# Autodesk Inventor assembly: YAxisMotor
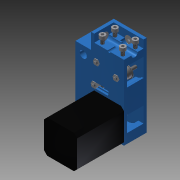
[picture p0: Inventor's stored thumbnail of the model, 180x180]
Saved by Autodesk Inventor 2015 (Build 190159000, 159)
## iProperties
Created: 2014-08-15
Part Number: YAxisMotor
Document SubType Name: Assembly
Designer: t_clevj
Author: t_clevj
## Documents named in this file (13)
- C:\Users\Jack\ownCloud\Projects\CoreXY\InventorModel\YAxis\YAxisMotor.iam
- C:\Users\Jack\ownCloud\Projects\CoreXY\InventorModel\YAxis\YAxisMotor\YMotorBlockLeft.ipt
- C:\Users\Jack\ownCloud\Projects\CoreXY\InventorModel\YAxis\YAxisMotor\YMotorCapLeft.ipt
- C:\Users\Jack\ownCloud\Projects\CoreXY\InventorModel\Hardware\Bolts\SHCS\SHCS4\SHCS4x30.ipt
- C:\Users\Jack\ownCloud\Projects\CoreXY\InventorModel\Hardware\Bolts\SHCS\SHCS3\SHCS3x8.ipt
- C:\Users\Jack\ownCloud\Projects\CoreXY\InventorModel\Hardware\Bolts\SHCS\SHCS5\SHCS5x10.ipt
- C:\Users\Jack\ownCloud\Projects\CoreXY\InventorModel\Hardware\Bearing\BearingRadialBall\BearingRadialBallF624zz.ipt
- C:\Users\Jack\ownCloud\Projects\CoreXY\InventorModel\Hardware\Wahsers\M4Washer.ipt
- C:\Users\Jack\ownCloud\Projects\CoreXY\InventorModel\Hardware\Nuts\Nut4.ipt
- C:\Users\Jack\ownCloud\Projects\CoreXY\InventorModel\Electronics\Motors\StepperMotorNema17.ipt
- C:\Users\Jack\ownCloud\Projects\CoreXY\InventorModel\Hardware\Bolts\SHCS\SHCS4\SHCS4x15.ipt
- C:\Users\Jack\ownCloud\Projects\CoreXY\InventorModel\Hardware\Bolts\FHS\FHS5\5x10FHS.ipt
- C:\Users\Jack\ownCloud\Projects\CoreXY\InventorModel\Hardware\Belt\PulleyGT2x20tx5mmBore.ipt
## Components (38 placed, 12 different names)
1. YMotorBlockLeft:1 — Mate:1, Mate:4, Flush:3, Mate:5, Mate:6, Mate:7, Mate:8, Slider:2, Mate:9, Mate:10, Mate:11, Mate:12, Mate:13, Mate:14, Mate:15, Mate:16, Mate:17, Mate:18, Mate:19, Mate:20, Mate:21, Mate:22, Mate:30, Mate:38, Mate:46, Angle:1, Mate:48, Angle:2, Mate:50, Angle:3, Mate:52, Mate:53, Mate:54, Angle:4, Angle:5, Angle:6, Angle:7, Mate:68, Mate:69, Mate:70, Mate:71, Mate:72, Mate:73, Flush:4, Flush:5, Mate:75
2. YMotorCapLeft:1 — Mate:1, Mate:6, Mate:56, Mate:57, Mate:58, Mate:59, Mate:60, Mate:61, Mate:62, Mate:63
3. SHCS4x30:3 — Mate:7, Mate:10, Mate:37, Mate:49
4. StepperMotorNema17:1 — Mate:53, Mate:54, Mate:55, Mate:74
5. 5x10FHS:1 — Mate:72, Flush:5
6. 5x10FHS:2 — Mate:73, Flush:4
7. PulleyGT2x20tx5mmBore:1 — Mate:74, Mate:75
8. Nut4:1 — Mate:47, Angle:1, Mate:48
9. Nut4:2 — Mate:49, Angle:2, Mate:50
10. Nut4:3 — Mate:51, Angle:3, Mate:52
11. M4Washer:1 — Mate:25, Mate:26
12. M4Washer:2 — Mate:27, Mate:28, Mate:29, Mate:30
13. M4Washer:3 — Mate:37
14. M4Washer:4 — Mate:38
15. M4Washer:5 — Mate:45
16. M4Washer:6 — Mate:46
17. SHCS4x30:5 — Slider:2, Mate:45, Mate:51
18. SHCS4x30:4 — Mate:8, Mate:9, Mate:29, Mate:47
19. BearingRadialBallF624zz:1 — Mate:23, Mate:24, Mate:25, Mate:26
20. BearingRadialBallF624zz:6 — Mate:23, Mate:24, Mate:27, Mate:28
21. BearingRadialBallF624zz:7
22. BearingRadialBallF624zz:8
23. BearingRadialBallF624zz:9
24. BearingRadialBallF624zz:10
25. SHCS5x10:2 — Mate:20, Mate:21
26. SHCS5x10:1 — Mate:19, Mate:22
27. SHCS3x8:3 — Mate:14, Mate:17
28. SHCS3x8:1 — Mate:12, Mate:18
29. SHCS3x8:2 — Mate:13, Mate:16
30. SHCS3x8:4 — Mate:11, Mate:15, Mate:55
31. SHCS4x15:1 — Mate:59, Mate:61, Mate:65
32. SHCS4x15:2 — Mate:58, Mate:62, Mate:67
33. SHCS4x15:3 — Mate:57, Mate:60, Mate:64
34. SHCS4x15:4 — Mate:56, Mate:63, Mate:66
35. Nut4:4 — Mate:66, Angle:6, Mate:70
36. Nut4:5 — Mate:67, Angle:7, Mate:71
37. Nut4:6 — Mate:64, Angle:5, Mate:69
38. Nut4:7 — Mate:65, Angle:4, Mate:68
## Relationships (84: Mate 73, Angle 7, Flush 3, TranslationJoint 1)
- Mate:1: YMotorBlockLeft:1 ↔ YMotorCapLeft:1
- Mate:4: YMotorBlockLeft:1
- Flush:3: YMotorBlockLeft:1
- Mate:5: YMotorBlockLeft:1
- Mate:6: YMotorBlockLeft:1 ↔ YMotorCapLeft:1
- Mate:7: YMotorBlockLeft:1 ↔ SHCS4x30:3
- Mate:8: YMotorBlockLeft:1 ↔ SHCS4x30:4
- Slider:2 [TranslationJoint]: YMotorBlockLeft:1 ↔ SHCS4x30:5
- Mate:9: YMotorBlockLeft:1 ↔ SHCS4x30:4
- Mate:10: YMotorBlockLeft:1 ↔ SHCS4x30:3
- Mate:11: YMotorBlockLeft:1 ↔ SHCS3x8:4
- Mate:12: YMotorBlockLeft:1 ↔ SHCS3x8:1
- Mate:13: YMotorBlockLeft:1 ↔ SHCS3x8:2
- Mate:14: YMotorBlockLeft:1 ↔ SHCS3x8:3
- Mate:15: YMotorBlockLeft:1 ↔ SHCS3x8:4
- Mate:16: YMotorBlockLeft:1 ↔ SHCS3x8:2
- Mate:17: YMotorBlockLeft:1 ↔ SHCS3x8:3
- Mate:18: YMotorBlockLeft:1 ↔ SHCS3x8:1
- Mate:19: YMotorBlockLeft:1 ↔ SHCS5x10:1
- Mate:20: YMotorBlockLeft:1 ↔ SHCS5x10:2
- Mate:21: YMotorBlockLeft:1 ↔ SHCS5x10:2
- Mate:22: YMotorBlockLeft:1 ↔ SHCS5x10:1
- Mate:23: BearingRadialBallF624zz:1 ↔ BearingRadialBallF624zz:6
- Mate:24: BearingRadialBallF624zz:1 ↔ BearingRadialBallF624zz:6
- Mate:25: M4Washer:1 ↔ BearingRadialBallF624zz:1
- Mate:26: M4Washer:1 ↔ BearingRadialBallF624zz:1
- Mate:27: M4Washer:2 ↔ BearingRadialBallF624zz:6
- Mate:28: M4Washer:2 ↔ BearingRadialBallF624zz:6
- Mate:29: M4Washer:2 ↔ SHCS4x30:4
- Mate:30: YMotorBlockLeft:1 ↔ M4Washer:2
- [Mate]: BearingRadialBallF624zz:7 ↔ BearingRadialBallF624zz:8
- [Mate]: BearingRadialBallF624zz:7 ↔ BearingRadialBallF624zz:8
- [Mate]: M4Washer:3 ↔ BearingRadialBallF624zz:7
- [Mate]: M4Washer:3 ↔ BearingRadialBallF624zz:7
- [Mate]: M4Washer:4 ↔ BearingRadialBallF624zz:8
- [Mate]: M4Washer:4 ↔ BearingRadialBallF624zz:8
- Mate:37: SHCS4x30:3 ↔ M4Washer:3
- Mate:38: YMotorBlockLeft:1 ↔ M4Washer:4
- [Mate]: BearingRadialBallF624zz:9 ↔ BearingRadialBallF624zz:10
- [Mate]: BearingRadialBallF624zz:9 ↔ BearingRadialBallF624zz:10
- [Mate]: M4Washer:5 ↔ BearingRadialBallF624zz:9
- [Mate]: M4Washer:5 ↔ BearingRadialBallF624zz:9
- [Mate]: M4Washer:6 ↔ BearingRadialBallF624zz:10
- [Mate]: M4Washer:6 ↔ BearingRadialBallF624zz:10
- Mate:45: M4Washer:5 ↔ SHCS4x30:5
- Mate:46: YMotorBlockLeft:1 ↔ M4Washer:6
- Mate:47: Nut4:1 ↔ SHCS4x30:4
- Angle:1 (0 deg): YMotorBlockLeft:1 ↔ Nut4:1
- Mate:48: YMotorBlockLeft:1 ↔ Nut4:1
- Mate:49: SHCS4x30:3 ↔ Nut4:2
- Angle:2 (0 deg): YMotorBlockLeft:1 ↔ Nut4:2
- Mate:50: YMotorBlockLeft:1 ↔ Nut4:2
- Mate:51: Nut4:3 ↔ SHCS4x30:5
- Angle:3 (0 deg): YMotorBlockLeft:1 ↔ Nut4:3
- Mate:52: YMotorBlockLeft:1 ↔ Nut4:3
- Mate:53: YMotorBlockLeft:1 ↔ StepperMotorNema17:1
- Mate:54: YMotorBlockLeft:1 ↔ StepperMotorNema17:1
- Mate:55: StepperMotorNema17:1 ↔ SHCS3x8:4
- Mate:56: YMotorCapLeft:1 ↔ SHCS4x15:4
- Mate:57: YMotorCapLeft:1 ↔ SHCS4x15:3
- Mate:58: YMotorCapLeft:1 ↔ SHCS4x15:2
- Mate:59: YMotorCapLeft:1 ↔ SHCS4x15:1
- Mate:60: YMotorCapLeft:1 ↔ SHCS4x15:3
- Mate:61: YMotorCapLeft:1 ↔ SHCS4x15:1
- Mate:62: YMotorCapLeft:1 ↔ SHCS4x15:2
- Mate:63: YMotorCapLeft:1 ↔ SHCS4x15:4
- Mate:64: SHCS4x15:3 ↔ Nut4:6
- Mate:65: SHCS4x15:1 ↔ Nut4:7
- Mate:66: SHCS4x15:4 ↔ Nut4:4
- Mate:67: SHCS4x15:2 ↔ Nut4:5
- Angle:4 (0 deg): YMotorBlockLeft:1 ↔ Nut4:7
- Angle:5 (0 deg): YMotorBlockLeft:1 ↔ Nut4:6
- Angle:6 (0 deg): YMotorBlockLeft:1 ↔ Nut4:4
- Angle:7 (0 deg): YMotorBlockLeft:1 ↔ Nut4:5
- Mate:68: YMotorBlockLeft:1 ↔ Nut4:7
- Mate:69: YMotorBlockLeft:1 ↔ Nut4:6
- Mate:70: YMotorBlockLeft:1 ↔ Nut4:4
- Mate:71: YMotorBlockLeft:1 ↔ Nut4:5
- Mate:72: YMotorBlockLeft:1 ↔ 5x10FHS:1
- Mate:73: YMotorBlockLeft:1 ↔ 5x10FHS:2
- Flush:4: YMotorBlockLeft:1 ↔ 5x10FHS:2
- Flush:5: YMotorBlockLeft:1 ↔ 5x10FHS:1
- Mate:74: StepperMotorNema17:1 ↔ PulleyGT2x20tx5mmBore:1
- Mate:75 (1.3 mm): YMotorBlockLeft:1 ↔ PulleyGT2x20tx5mmBore:1
## Named parameters: d52_d44 = 0 mm, d53_d45 = 0 mm, d54_d46 = 0 mm, d55_d47 = 0 mm, d56_d48 = 0 mm, d57_d49 = 0 mm, d60_d44 = 0 mm, d61_d45 = 0 mm, d62_d46 = 0 mm, d63_d47 = 0 mm, d64_d48 = 0 mm, d65_d49 = 0 mm
